# Autodesk Inventor assembly: ミラー
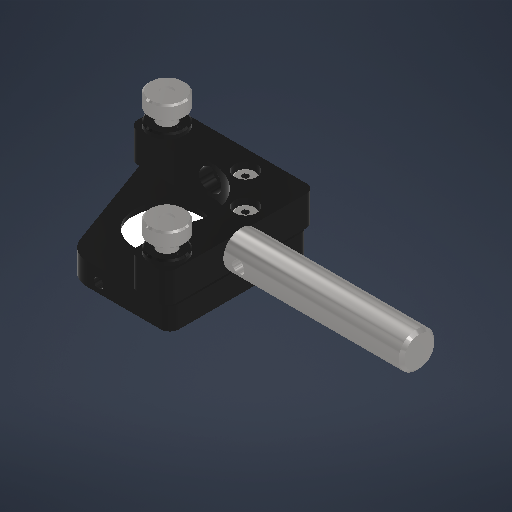
[picture p0: Inventor's stored thumbnail of the model, 512x512]
Saved by Autodesk Inventor 2026 (Build 300175050, 175E)
## iProperties
Created: 2025-07-10
Part Number: ミラー
Document SubType Name: Assembly
Designer: jin20
Author: jin20
## Documents named in this file (4)
- C:\Users\jin20\Documents\装置CAD\RamanSystem\Optics\ミラー.iam
- C:\Users\jin20\Documents\装置CAD\RamanSystem\Optics\ミラーマウント\ミラーマウント.iam
- C:\Users\jin20\Documents\装置CAD\RamanSystem\Optics\ミラー.ipt
- C:\Users\jin20\Documents\装置CAD\RamanSystem\Optics\ロッド\ロッド_60mm.ipt
## Components (3 placed, 3 different names)
1. ミラーマウント:1 [sub-assembly] — 挿入:1, 挿入:2
2. ミラー:1 — 挿入:1
3. ロッド_60mm:1 — 挿入:2
## Relationships (2: Insert 2)
- 挿入:1 [Insert]: ミラーマウント:1 ↔ ミラー:1
- 挿入:2 [Insert]: ミラーマウント:1 ↔ ロッド_60mm:1
